# Autodesk Inventor assembly: Assembly3
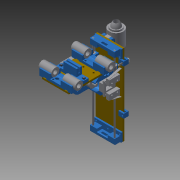
[picture p0: Inventor's stored thumbnail of the model, 180x180]
Saved by Autodesk Inventor 2013 SP2 (Build 170200200, 200)
## iProperties
Created: 2017-01-25
Part Number: Assembly3
Document SubType Name: Assembly
Designer: Herman de Vries
Mass: 50.9639 g
Surface Area: 318.396 cm^2
Volume: 50.9639 cm^3
Density: 1 g/cm^3
Author: Herman de Vries
## Documents named in this file (7)
- C:\Users\hdv\Dropbox\Projects\Inventor\PaintBot_3\Z Rail assy.iam
- C:\Users\hdv\Dropbox\Projects\Inventor\PaintBot_3\Z Rail.ipt
- C:\Users\hdv\Dropbox\Projects\Inventor\PaintBot_3\GT2 grip.ipt
- C:\Users\hdv\Dropbox\Projects\Inventor\PaintBot_3\Linear bearing 8mm.ipt
- C:\Users\hdv\Dropbox\Projects\Inventor\PaintBot_3\Linear bearing 8mm clamp.ipt
- C:\Users\hdv\Dropbox\Projects\Inventor\parts\P-BD000035 - Screw M3x10mm Hex Socket Head Cap SS ISO4762.ipt
- C:\Users\hdv\Dropbox\Projects\Inventor\PaintBot_3\z_axis\z axis.iam
## Components (11 placed, 6 different names)
1. Z Rail:1 — Mate:15, Flush:16, Flush:20, Mate:16, Flush:21, Mate:19, Flush:28, Insert:1, Insert:2
2. GT2 grip:1 — Mate:15, Flush:16, Flush:20
3. Linear bearing 8mm:1 — Mate:18, Flush:25
4. Linear bearing 8mm:2 — Mate:17, Flush:26
5. Linear bearing 8mm:3 — Mate:20, Flush:24
6. Linear bearing 8mm clamp:1 — Mate:16, Flush:21, Mate:17, Mate:18, Flush:22, Flush:25, Flush:26, Flush:28, Mate:22
7. Linear bearing 8mm clamp:2 — Mate:19, Flush:22, Mate:20, Flush:24, Mate:21, Flush:27, Mate:22
8. Linear bearing 8mm:4 — Mate:21, Flush:27
9. P-BD000035 - Screw M3x10mm Hex Socket Head Cap SS ISO4762:1 — Insert:1
10. P-BD000035 - Screw M3x10mm Hex Socket Head Cap SS ISO4762:2 — Insert:2
11. z axis:1 [sub-assembly]
## Relationships (22: Flush 11, Mate 9, Insert 2)
- Mate:15: Z Rail:1 ↔ GT2 grip:1
- Flush:16 (27 mm): Z Rail:1 ↔ GT2 grip:1
- Flush:20: Z Rail:1 ↔ GT2 grip:1
- Mate:16: Z Rail:1 ↔ Linear bearing 8mm clamp:1
- Flush:21 (-5 mm): Z Rail:1 ↔ Linear bearing 8mm clamp:1
- Mate:17: Linear bearing 8mm:2 ↔ Linear bearing 8mm clamp:1
- Mate:18: Linear bearing 8mm:1 ↔ Linear bearing 8mm clamp:1
- Mate:19: Z Rail:1 ↔ Linear bearing 8mm clamp:2
- Flush:22: Linear bearing 8mm clamp:1 ↔ Linear bearing 8mm clamp:2
- Mate:20: Linear bearing 8mm:3 ↔ Linear bearing 8mm clamp:2
- Flush:24: Linear bearing 8mm:3 ↔ Linear bearing 8mm clamp:2
- Flush:25: Linear bearing 8mm:1 ↔ Linear bearing 8mm clamp:1
- Flush:26: Linear bearing 8mm:2 ↔ Linear bearing 8mm clamp:1
- Mate:21: Linear bearing 8mm clamp:2 ↔ Linear bearing 8mm:4
- Flush:27: Linear bearing 8mm clamp:2 ↔ Linear bearing 8mm:4
- Flush:28: Z Rail:1 ↔ Linear bearing 8mm clamp:1
- Mate:22 (40 mm): Linear bearing 8mm clamp:1 ↔ Linear bearing 8mm clamp:2
- Insert:1: Z Rail:1 ↔ P-BD000035 - Screw M3x10mm Hex Socket Head Cap SS ISO4762:1
- Insert:2: Z Rail:1 ↔ P-BD000035 - Screw M3x10mm Hex Socket Head Cap SS ISO4762:2
- [Mate]: Z Rail:1 ↔ z axis:1
- [Flush] (-10 mm): Z Rail:1 ↔ z axis:1
- [Flush] (6 mm): Z Rail:1 ↔ z axis:1
